# Autodesk Inventor assembly: gearbox_MIR
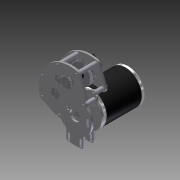
[picture p0: Inventor's stored thumbnail of the model, 180x180]
Saved by Autodesk Inventor 2012 (Build 160160000, 160)
## iProperties
Created: 2012-01-30
Part Number: gearbox_MIR
Document SubType Name: Assembly
Designer: Antonella Wilby
Author: Antonella Wilby
## Documents named in this file (42)
- C:\Users\Antonella\Documents\GCC Robotics 2012 - Mechanical\Robot 2.0\Drive Train\Gearbox\gearbox_MIR.iam
- C:\Users\Antonella\Documents\GCC Robotics 2012 - Mechanical\Robot 2.0\Drive Train\MY1020 Motor\my1020_motor_MIR.iam
- C:\Users\Antonella\Documents\GCC Robotics 2012 - Mechanical\Robot 2.0\Drive Train\Gearbox\standoff 2in_MIR.ipt
- C:\Users\Antonella\Documents\GCC Robotics 2012 - Mechanical\Robot 2.0\Drive Train\Gearbox\standoff 1.25in_MIR.ipt
- C:\Users\Antonella\Documents\GCC Robotics 2012 - Mechanical\Robot 2.0\Drive Train\Gearbox\fr8-zz_MIR.ipt
- C:\Users\Antonella\Documents\GCC Robotics 2012 - Mechanical\Robot 2.0\Drive Train\Gearbox\standoff 4.25in_MIR.ipt
- C:\Users\Antonella\Documents\GCC Robotics 2012 - Mechanical\Robot 2.0\Drive Train\Gearbox\fr6-zz_MIR.ipt
- C:\Users\Antonella\Documents\GCC Robotics 2012 - Mechanical\Robot 2.0\Drive Train\Gearbox\output_shaft_MIR.ipt
- C:\Users\Antonella\Documents\GCC Robotics 2012 - Mechanical\Robot 2.0\Drive Train\Gearbox\spur gear - 24t x 20dp x dd shaft_MIR.ipt
- C:\Users\Antonella\Documents\GCC Robotics 2012 - Mechanical\Robot 2.0\Drive Train\Gearbox\encoder mount_MIR.ipt
- C:\Users\Antonella\Documents\GCC Robotics 2012 - Mechanical\Robot 2.0\Electrical\encoder_MIR.ipt
- C:\Users\Antonella\Documents\GCC Robotics 2012 - Mechanical\Robot 2.0\Drive Train\Gearbox\spur gear -  60t x 20dp x 0.5 hexbore_MIR.ipt
- C:\Users\Antonella\Documents\GCC Robotics 2012 - Mechanical\Robot 2.0\Drive Train\Gearbox\spur gear - 14t x 20dp x 0.375 hexbore_MIR.ipt
- C:\Users\Antonella\Documents\GCC Robotics 2012 - Mechanical\Robot 2.0\Drive Train\Gearbox\output sprocket - No. 25 x 16t_MIR.ipt
- C:\Users\Antonella\Documents\GCC Robotics 2012 - Mechanical\Robot 2.0\Drive Train\Gearbox\spur gear - 50t x 20dp x 0.5 hexbore_MIR.ipt
- C:\Users\Antonella\Documents\GCC Robotics 2012 - Mechanical\Robot 2.0\Drive Train\Gearbox\spur gear - 50t x 20dp x 0.375 hexbore_MIR.ipt
- C:\Users\Antonella\Documents\GCC Robotics 2012 - Mechanical\Robot 2.0\Drive Train\Gearbox\shaft - step down No. 2 - 0.375 hex_MIR.ipt
- C:\Users\Antonella\Documents\GCC Robotics 2012 - Mechanical\Robot 2.0\Drive Train\Gearbox\shaft - step down No. 1 - 0.5 hex_MIR.ipt
- C:\Users\Antonella\Documents\GCC Robotics 2012 - Mechanical\Robot 2.0\Drive Train\Gearbox\spur gear - 19t x 20dp x 0.375 hexbore_MIR.ipt
- C:\Users\Antonella\Documents\GCC Robotics 2012 - Mechanical\Robot 2.0\Drive Train\Gearbox\back plate_MIR.ipt
- C:\Users\Antonella\Documents\GCC Robotics 2012 - Mechanical\Robot 2.0\Drive Train\Gearbox\motor plate_MIR.ipt
- C:\Users\Antonella\Documents\GCC Robotics 2012 - Mechanical\Robot 2.0\Drive Train\Gearbox\front plate_MIR.ipt
- C:\Users\Antonella\Documents\GCC Robotics 2012 - Mechanical\Robot 2.0\Drive Train\Gearbox\fr4_MIR.ipt
- C:\Users\Antonella\Documents\GCC Robotics 2012 - Mechanical\Robot 2.0\Drive Train\Gearbox\idler gear shaft_MIR.ipt
- C:\Users\Antonella\Documents\GCC Robotics 2012 - Mechanical\Robot 2.0\Drive Train\Gearbox\e-clip .375in shaft_MIR.ipt
- C:\Users\Antonella\Documents\GCC Robotics 2012 - Mechanical\Robot 2.0\Drive Train\Gearbox\e-clip .5in shaft_MIR.ipt
- C:\Users\Antonella\Documents\GCC Robotics 2012 - Mechanical\Robot 2.0\Drive Train\Gearbox\gearbox\Design Accelerator\Bolted Connection1_MIR.iam
- C:\Users\Antonella\Documents\GCC Robotics 2012 - Mechanical\Robot 2.0\Drive Train\Gearbox\gearbox\Design Accelerator\Bolted Connection2_MIR.iam
- C:\Users\Antonella\Documents\GCC Robotics 2012 - Mechanical\Robot 2.0\Drive Train\Gearbox\gearbox\Design Accelerator\Bolted Connection4_MIR.iam
- C:\Users\Antonella\Documents\GCC Robotics 2012 - Mechanical\Robot 2.0\Drive Train\Gearbox\gearbox\Design Accelerator\Bolted Connection5_MIR.iam
- C:\Users\Antonella\Documents\GCC Robotics 2012 - Mechanical\Robot 2.0\Drive Train\Gearbox\gearbox\Design Accelerator\Bolted Connection7_MIR.iam
- C:\Users\Antonella\Documents\GCC Robotics 2012 - Mechanical\Robot 2.0\Drive Train\Gearbox\gearbox\Design Accelerator\Bolted Connection8_MIR.iam
- C:\Users\Antonella\Documents\GCC Robotics 2012 - Mechanical\Robot 2.0\Drive Train\Gearbox\gearbox\Design Accelerator\Bolted Connection9_MIR.iam
- C:\Users\Antonella\Documents\GCC Robotics 2012 - Mechanical\Robot 2.0\Drive Train\Gearbox\gearbox\Design Accelerator\Bolted Connection10_MIR.iam
- C:\Users\Antonella\Documents\GCC Robotics 2012 - Mechanical\Robot 2.0\Drive Train\Gearbox\gearbox\Design Accelerator\Bolted Connection12_MIR.iam
- C:\Users\Antonella\Documents\GCC Robotics 2012 - Mechanical\Robot 2.0\Drive Train\Gearbox\gearbox\Design Accelerator\Bolted Connection13_MIR.iam
- C:\Users\Antonella\Documents\GCC Robotics 2012 - Mechanical\Robot 2.0\Drive Train\Gearbox\gearbox\Design Accelerator\Bolted Connection14_MIR.iam
- C:\Users\Antonella\Documents\GCC Robotics 2012 - Mechanical\Robot 2.0\Drive Train\Gearbox\gearbox\Design Accelerator\Bolted Connection15_MIR.iam
- C:\Users\Antonella\Documents\GCC Robotics 2012 - Mechanical\Robot 2.0\Drive Train\Gearbox\gearbox\Design Accelerator\Bolted Connection16_MIR.iam
- C:\Users\Antonella\Documents\GCC Robotics 2012 - Mechanical\Robot 2.0\Drive Train\Gearbox\gearbox\Design Accelerator\Bolted Connection17_MIR.iam
- C:\Users\Antonella\Documents\GCC Robotics 2012 - Mechanical\Robot 2.0\Drive Train\Gearbox\gearbox\Design Accelerator\Bolted Connection18_MIR.iam
- C:\Users\Antonella\Documents\GCC Robotics 2012 - Mechanical\Robot 2.0\Drive Train\Gearbox\gearbox\Design Accelerator\Bolted Connection19_MIR.iam
## Components (58 placed, 41 different names)
1. my1020_motor_MIR:1 [sub-assembly] — Flush:1, Mate:40, Mate:39, Mate:82, Mate:118, Mate:108, Mate:107
2. standoff 2in_MIR:1 — Mate:123, Mate:122
3. standoff 2in_MIR:2 — Mate:120, Mate:119, Mate:121
4. standoff 1.25in_MIR:1 — Mate:131, Mate:130
5. standoff 1.25in_MIR:2 — Mate:129, Mate:128
6. fr8-zz_MIR:1 — Mate:100, Mate:99, Mate:94, Mate:93
7. fr8-zz_MIR:2 — Mate:136, Mate:135
8. standoff 4.25in_MIR:1 — Mate:127, Mate:126, Mate:132
9. standoff 4.25in_MIR:2 — Mate:125, Mate:124, Mate:134
10. fr6-zz_MIR:1 — Mate:102, Mate:101, Mate:106, Mate:96, Mate:95
11. fr6-zz_MIR:2 — Mate:104, Mate:103, Mate:98, Mate:97
12. fr6-zz_MIR:3 — Mate:138, Mate:137
13. output_shaft_MIR:1 — Mate:100, Mate:99, Flush:76, Mate:77, Mate:58, Flush:3, Mate:165, Mate:164, Mate:167, Mate:166
14. spur gear - 24t x 20dp x dd shaft_MIR:1 — Flush:1, Mate:40, Mate:39
15. encoder mount_MIR:1 — Flush:2, Mate:49, Mate:48, Mate:92, Mate:84, Mate:83
16. encoder_MIR:1 — Flush:2, Mate:49, Mate:48
17. spur gear -  60t x 20dp x 0.5 hexbore_MIR:1 — Mate:70, Mate:69, Mate:116
18. spur gear - 14t x 20dp x 0.375 hexbore_MIR:1 — Flush:80, Mate:80, Flush:63, Mate:64
19. output sprocket - No. 25 x 16t_MIR:1 — Flush:76, Mate:77, Mate:203
20. spur gear - 50t x 20dp x 0.5 hexbore_MIR:1 — Flush:80, Mate:58, Flush:3
21. spur gear - 50t x 20dp x 0.375 hexbore_MIR:1 — Mate:80, Mate:66, Mate:65, Flush:79
22. shaft - step down No. 2 - 0.375 hex_MIR:1 — Mate:104, Mate:103, Flush:63, Mate:66, Mate:65, Mate:64, Mate:161, Mate:160, Mate:169, Mate:168
23. shaft - step down No. 1 - 0.5 hex_MIR:1 — Mate:102, Mate:101, Mate:70, Mate:69, Flush:78, Mate:79, Mate:170, Mate:156, Mate:159, Mate:158
24. spur gear - 19t x 20dp x 0.375 hexbore_MIR:1 — Mate:106, Flush:79, Flush:78, Mate:79
25. fr8-zz_MIR:3 — Mate:203, Mate:140, Mate:139
26. back plate_MIR:1 — Mate:127, Mate:126, Mate:125, Mate:124, Mate:123, Mate:122, Mate:120, Mate:119, Mate:98, Mate:97, Mate:96, Mate:95, Mate:94, Mate:93, Mate:92, Mate:84, Mate:83, Mate:82, Mate:117, Mate:151, Mate:150, Mate:153, Mate:152, Mate:184, Mate:183, Mate:186, Mate:185, Mate:188, Mate:187, Mate:190, Mate:189
27. motor plate_MIR:1 — Mate:131, Mate:130, Mate:129, Mate:128, Mate:121, Mate:118, Mate:117, Mate:116, Mate:108, Mate:107, Mate:142, Mate:141, Mate:172, Mate:171, Mate:174, Mate:173, Mate:176, Mate:175, Mate:178, Mate:177, Mate:180, Mate:179, Mate:182, Mate:181
28. front plate_MIR:1 — Mate:140, Mate:139, Mate:138, Mate:137, Mate:136, Mate:135, Mate:134, Mate:132, Mate:144, Mate:143, Mate:192, Mate:191, Mate:194, Mate:193, Mate:196, Mate:195, Mate:198, Mate:197, Mate:200, Mate:199, Mate:202, Mate:201
29. spur gear - 14t x 20dp x 0.375 hexbore_MIR:2 — Mate:149, Flush:147, Mate:148
30. fr4_MIR:1 — Mate:149, Mate:142, Mate:141, Mate:146, Mate:145
31. fr4_MIR:2 — Mate:144, Mate:143
32. idler gear shaft_MIR:1 — Flush:147, Mate:148, Mate:146, Mate:145
33. standoff 4.25in_MIR:3 — Mate:151, Mate:150
34. standoff 4.25in_MIR:4 — Mate:153, Mate:152
35. e-clip .375in shaft_MIR:1
36. e-clip .5in shaft_MIR:1 — Mate:170, Mate:156
37. e-clip .5in shaft_MIR:2 — Mate:159, Mate:158
38. e-clip .375in shaft_MIR:2
39. e-clip .375in shaft_MIR:3 — Mate:161, Mate:160
40. e-clip .375in shaft_MIR:4 — Mate:169, Mate:168
41. e-clip .5in shaft_MIR:3 — Mate:165, Mate:164
42. e-clip .5in shaft_MIR:4 — Mate:167, Mate:166
43. Bolted Connection1_MIR:1 [sub-assembly] — Mate:172, Mate:171
44. Bolted Connection2_MIR:1 [sub-assembly] — Mate:174, Mate:173
45. Bolted Connection4_MIR:1 [sub-assembly] — Mate:176, Mate:175
46. Bolted Connection5_MIR:1 [sub-assembly] — Mate:178, Mate:177
47. Bolted Connection7_MIR:1 [sub-assembly] — Mate:180, Mate:179
48. Bolted Connection8_MIR:1 [sub-assembly] — Mate:182, Mate:181
49. Bolted Connection9_MIR:1 [sub-assembly] — Mate:184, Mate:183
50. Bolted Connection10_MIR:1 [sub-assembly] — Mate:186, Mate:185
51. Bolted Connection12_MIR:1 [sub-assembly] — Mate:188, Mate:187
52. Bolted Connection13_MIR:1 [sub-assembly] — Mate:190, Mate:189
53. Bolted Connection14_MIR:1 [sub-assembly] — Mate:192, Mate:191
54. Bolted Connection15_MIR:1 [sub-assembly] — Mate:194, Mate:193
55. Bolted Connection16_MIR:1 [sub-assembly] — Mate:196, Mate:195
56. Bolted Connection17_MIR:1 [sub-assembly] — Mate:198, Mate:197
57. Bolted Connection18_MIR:1 [sub-assembly] — Mate:200, Mate:199
58. Bolted Connection19_MIR:1 [sub-assembly] — Mate:202, Mate:201
## Relationships (122: Mate 97, Flush 25)
- Mate:100: fr8-zz_MIR:1 ↔ output_shaft_MIR:1
- Mate:99: fr8-zz_MIR:1 ↔ output_shaft_MIR:1
- Flush:1 (1.5875 mm): my1020_motor_MIR:1 ↔ spur gear - 24t x 20dp x dd shaft_MIR:1
- Mate:40: my1020_motor_MIR:1 ↔ spur gear - 24t x 20dp x dd shaft_MIR:1
- Mate:39: my1020_motor_MIR:1 ↔ spur gear - 24t x 20dp x dd shaft_MIR:1
- Flush:2: encoder mount_MIR:1 ↔ encoder_MIR:1
- Mate:49: encoder mount_MIR:1 ↔ encoder_MIR:1
- Mate:48: encoder mount_MIR:1 ↔ encoder_MIR:1
- Flush:76: output_shaft_MIR:1 ↔ output sprocket - No. 25 x 16t_MIR:1
- Mate:77: output_shaft_MIR:1 ↔ output sprocket - No. 25 x 16t_MIR:1
- Flush:80 (-2.8575 mm): spur gear - 14t x 20dp x 0.375 hexbore_MIR:1 ↔ spur gear - 50t x 20dp x 0.5 hexbore_MIR:1
- Mate:58: output_shaft_MIR:1 ↔ spur gear - 50t x 20dp x 0.5 hexbore_MIR:1
- Flush:3: output_shaft_MIR:1 ↔ spur gear - 50t x 20dp x 0.5 hexbore_MIR:1
- Mate:80: spur gear - 14t x 20dp x 0.375 hexbore_MIR:1 ↔ spur gear - 50t x 20dp x 0.375 hexbore_MIR:1
- Mate:104: fr6-zz_MIR:2 ↔ shaft - step down No. 2 - 0.375 hex_MIR:1
- Mate:103: fr6-zz_MIR:2 ↔ shaft - step down No. 2 - 0.375 hex_MIR:1
- Flush:63: spur gear - 14t x 20dp x 0.375 hexbore_MIR:1 ↔ shaft - step down No. 2 - 0.375 hex_MIR:1
- Mate:66: spur gear - 50t x 20dp x 0.375 hexbore_MIR:1 ↔ shaft - step down No. 2 - 0.375 hex_MIR:1
- Mate:65: spur gear - 50t x 20dp x 0.375 hexbore_MIR:1 ↔ shaft - step down No. 2 - 0.375 hex_MIR:1
- Mate:64: spur gear - 14t x 20dp x 0.375 hexbore_MIR:1 ↔ shaft - step down No. 2 - 0.375 hex_MIR:1
- Mate:102: fr6-zz_MIR:1 ↔ shaft - step down No. 1 - 0.5 hex_MIR:1
- Mate:101: fr6-zz_MIR:1 ↔ shaft - step down No. 1 - 0.5 hex_MIR:1
- Mate:70: spur gear -  60t x 20dp x 0.5 hexbore_MIR:1 ↔ shaft - step down No. 1 - 0.5 hex_MIR:1
- Mate:69: spur gear -  60t x 20dp x 0.5 hexbore_MIR:1 ↔ shaft - step down No. 1 - 0.5 hex_MIR:1
- Mate:106: fr6-zz_MIR:1 ↔ spur gear - 19t x 20dp x 0.375 hexbore_MIR:1
- Flush:79 (-2.8765 mm): spur gear - 50t x 20dp x 0.375 hexbore_MIR:1 ↔ spur gear - 19t x 20dp x 0.375 hexbore_MIR:1
- Flush:78: shaft - step down No. 1 - 0.5 hex_MIR:1 ↔ spur gear - 19t x 20dp x 0.375 hexbore_MIR:1
- Mate:79: shaft - step down No. 1 - 0.5 hex_MIR:1 ↔ spur gear - 19t x 20dp x 0.375 hexbore_MIR:1
- Mate:203: output sprocket - No. 25 x 16t_MIR:1 ↔ fr8-zz_MIR:3
- Mate:127: standoff 4.25in_MIR:1 ↔ back plate_MIR:1
- Mate:126: standoff 4.25in_MIR:1 ↔ back plate_MIR:1
- Mate:125: standoff 4.25in_MIR:2 ↔ back plate_MIR:1
- Mate:124: standoff 4.25in_MIR:2 ↔ back plate_MIR:1
- Mate:123: standoff 2in_MIR:1 ↔ back plate_MIR:1
- Mate:122: standoff 2in_MIR:1 ↔ back plate_MIR:1
- Mate:120: standoff 2in_MIR:2 ↔ back plate_MIR:1
- Mate:119: standoff 2in_MIR:2 ↔ back plate_MIR:1
- Mate:98: fr6-zz_MIR:2 ↔ back plate_MIR:1
- Mate:97: fr6-zz_MIR:2 ↔ back plate_MIR:1
- Mate:96: fr6-zz_MIR:1 ↔ back plate_MIR:1
- Mate:95: fr6-zz_MIR:1 ↔ back plate_MIR:1
- Mate:94: fr8-zz_MIR:1 ↔ back plate_MIR:1
- Mate:93: fr8-zz_MIR:1 ↔ back plate_MIR:1
- Mate:92: encoder mount_MIR:1 ↔ back plate_MIR:1
- Mate:84: encoder mount_MIR:1 ↔ back plate_MIR:1
- Mate:83: encoder mount_MIR:1 ↔ back plate_MIR:1
- Mate:82: my1020_motor_MIR:1 ↔ back plate_MIR:1
- Mate:131: standoff 1.25in_MIR:1 ↔ motor plate_MIR:1
- Mate:130: standoff 1.25in_MIR:1 ↔ motor plate_MIR:1
- Mate:129: standoff 1.25in_MIR:2 ↔ motor plate_MIR:1
- Mate:128: standoff 1.25in_MIR:2 ↔ motor plate_MIR:1
- Mate:121: standoff 2in_MIR:2 ↔ motor plate_MIR:1
- Mate:118: my1020_motor_MIR:1 ↔ motor plate_MIR:1
- Mate:117: back plate_MIR:1 ↔ motor plate_MIR:1
- Mate:116 (4.7625 mm): spur gear -  60t x 20dp x 0.5 hexbore_MIR:1 ↔ motor plate_MIR:1
- Mate:108: my1020_motor_MIR:1 ↔ motor plate_MIR:1
- Mate:107: my1020_motor_MIR:1 ↔ motor plate_MIR:1
- Mate:140: fr8-zz_MIR:3 ↔ front plate_MIR:1
- Mate:139: fr8-zz_MIR:3 ↔ front plate_MIR:1
- Mate:138: fr6-zz_MIR:3 ↔ front plate_MIR:1
- Mate:137: fr6-zz_MIR:3 ↔ front plate_MIR:1
- Mate:136: fr8-zz_MIR:2 ↔ front plate_MIR:1
- Mate:135: fr8-zz_MIR:2 ↔ front plate_MIR:1
- Mate:134: standoff 4.25in_MIR:2 ↔ front plate_MIR:1
- Mate:132: standoff 4.25in_MIR:1 ↔ front plate_MIR:1
- Mate:149: spur gear - 14t x 20dp x 0.375 hexbore_MIR:2 ↔ fr4_MIR:1
- Mate:142: motor plate_MIR:1 ↔ fr4_MIR:1
- Mate:141: motor plate_MIR:1 ↔ fr4_MIR:1
- Mate:144: front plate_MIR:1 ↔ fr4_MIR:2
- Mate:143: front plate_MIR:1 ↔ fr4_MIR:2
- Flush:147: spur gear - 14t x 20dp x 0.375 hexbore_MIR:2 ↔ idler gear shaft_MIR:1
- Mate:148: spur gear - 14t x 20dp x 0.375 hexbore_MIR:2 ↔ idler gear shaft_MIR:1
- Mate:146: fr4_MIR:1 ↔ idler gear shaft_MIR:1
- Mate:145: fr4_MIR:1 ↔ idler gear shaft_MIR:1
- Mate:151: back plate_MIR:1 ↔ standoff 4.25in_MIR:3
- Mate:150: back plate_MIR:1 ↔ standoff 4.25in_MIR:3
- Mate:153: back plate_MIR:1 ↔ standoff 4.25in_MIR:4
- Mate:152: back plate_MIR:1 ↔ standoff 4.25in_MIR:4
- Mate:170: shaft - step down No. 1 - 0.5 hex_MIR:1 ↔ e-clip .5in shaft_MIR:1
- Mate:156: shaft - step down No. 1 - 0.5 hex_MIR:1 ↔ e-clip .5in shaft_MIR:1
- Mate:159: shaft - step down No. 1 - 0.5 hex_MIR:1 ↔ e-clip .5in shaft_MIR:2
- Mate:158: shaft - step down No. 1 - 0.5 hex_MIR:1 ↔ e-clip .5in shaft_MIR:2
- Mate:161: shaft - step down No. 2 - 0.375 hex_MIR:1 ↔ e-clip .375in shaft_MIR:3
- Mate:160: shaft - step down No. 2 - 0.375 hex_MIR:1 ↔ e-clip .375in shaft_MIR:3
- Mate:169: shaft - step down No. 2 - 0.375 hex_MIR:1 ↔ e-clip .375in shaft_MIR:4
- Mate:168: shaft - step down No. 2 - 0.375 hex_MIR:1 ↔ e-clip .375in shaft_MIR:4
- Mate:165: output_shaft_MIR:1 ↔ e-clip .5in shaft_MIR:3
- Mate:164: output_shaft_MIR:1 ↔ e-clip .5in shaft_MIR:3
- Mate:167: output_shaft_MIR:1 ↔ e-clip .5in shaft_MIR:4
- Mate:166: output_shaft_MIR:1 ↔ e-clip .5in shaft_MIR:4
- Mate:172: motor plate_MIR:1 ↔ Bolted Connection1_MIR:1
- Mate:171 [Flush]: motor plate_MIR:1 ↔ Bolted Connection1_MIR:1
- Mate:174: motor plate_MIR:1 ↔ Bolted Connection2_MIR:1
- Mate:173 [Flush]: motor plate_MIR:1 ↔ Bolted Connection2_MIR:1
- Mate:176: motor plate_MIR:1 ↔ Bolted Connection4_MIR:1
- Mate:175 [Flush]: motor plate_MIR:1 ↔ Bolted Connection4_MIR:1
- Mate:178: motor plate_MIR:1 ↔ Bolted Connection5_MIR:1
- Mate:177 [Flush]: motor plate_MIR:1 ↔ Bolted Connection5_MIR:1
- Mate:180: motor plate_MIR:1 ↔ Bolted Connection7_MIR:1
- Mate:179 [Flush]: motor plate_MIR:1 ↔ Bolted Connection7_MIR:1
- Mate:182: motor plate_MIR:1 ↔ Bolted Connection8_MIR:1
- Mate:181 [Flush]: motor plate_MIR:1 ↔ Bolted Connection8_MIR:1
- Mate:184: back plate_MIR:1 ↔ Bolted Connection9_MIR:1
- Mate:183 [Flush]: back plate_MIR:1 ↔ Bolted Connection9_MIR:1
- Mate:186: back plate_MIR:1 ↔ Bolted Connection10_MIR:1
- Mate:185 [Flush]: back plate_MIR:1 ↔ Bolted Connection10_MIR:1
- Mate:188: back plate_MIR:1 ↔ Bolted Connection12_MIR:1
- Mate:187 [Flush]: back plate_MIR:1 ↔ Bolted Connection12_MIR:1
- Mate:190: back plate_MIR:1 ↔ Bolted Connection13_MIR:1
- Mate:189 [Flush]: back plate_MIR:1 ↔ Bolted Connection13_MIR:1
- Mate:192: front plate_MIR:1 ↔ Bolted Connection14_MIR:1
- Mate:191 [Flush]: front plate_MIR:1 ↔ Bolted Connection14_MIR:1
- Mate:194: front plate_MIR:1 ↔ Bolted Connection15_MIR:1
- Mate:193 [Flush]: front plate_MIR:1 ↔ Bolted Connection15_MIR:1
- Mate:196: front plate_MIR:1 ↔ Bolted Connection16_MIR:1
- Mate:195 [Flush]: front plate_MIR:1 ↔ Bolted Connection16_MIR:1
- Mate:198: front plate_MIR:1 ↔ Bolted Connection17_MIR:1
- Mate:197 [Flush]: front plate_MIR:1 ↔ Bolted Connection17_MIR:1
- Mate:200: front plate_MIR:1 ↔ Bolted Connection18_MIR:1
- Mate:199 [Flush]: front plate_MIR:1 ↔ Bolted Connection18_MIR:1
- Mate:202: front plate_MIR:1 ↔ Bolted Connection19_MIR:1
- Mate:201 [Flush]: front plate_MIR:1 ↔ Bolted Connection19_MIR:1
